# Autodesk Inventor assembly: planetaryGearBox
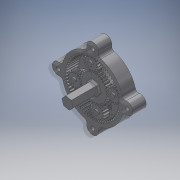
[picture p0: Inventor's stored thumbnail of the model, 180x180]
Saved by Autodesk Inventor 2019 (Build 230136000, 136)
## iProperties
Created: 2019-10-26
Part Number: planetaryGearBox
Document SubType Name: Assembly
Designer: test
Author: test
## Documents named in this file (6)
- C:\Users\test\Downloads\planetaryGearBox.iam
- C:\Users\test\Downloads\topPlateGB.ipt
- C:\Users\test\Downloads\planetaryGearMt2.ipt
- C:\Users\test\Downloads\RushGears_AP214_F3216.ipt
- C:\Users\test\Downloads\RushGears_AP214_F3232B.ipt
- C:\Users\test\Downloads\RushGears_AP214_F3264A.ipt
## Components (8 placed, 5 different names)
1. planetaryGearMt2:1 — Mate:1, Mate:2, Mate:3, Mate:4, Mate:5, Mate:6, Mate:7, Mate:8, Mate:10
2. RushGears_AP214_F3216:1 — Mate:3, Flush:1
3. RushGears_AP214_F3216:2 — Mate:5, Flush:4
4. RushGears_AP214_F3216:3 — Mate:6, Flush:2
5. RushGears_AP214_F3216:4 — Mate:4, Flush:3
6. RushGears_AP214_F3232B:1 — Mate:7, Flush:1, Flush:2, Flush:3, Flush:4, Mate:8
7. RushGears_AP214_F3264A:1 — Mate:1, Mate:2, Mate:9, Mate:11
8. topPlateGB:2 — Mate:9, Mate:10, Mate:11
## Relationships (15: Mate 11, Flush 4)
- Mate:1: planetaryGearMt2:1 ↔ RushGears_AP214_F3264A:1
- Mate:2: planetaryGearMt2:1 ↔ RushGears_AP214_F3264A:1
- Mate:3: planetaryGearMt2:1 ↔ RushGears_AP214_F3216:1
- Mate:4: planetaryGearMt2:1 ↔ RushGears_AP214_F3216:4
- Mate:5: planetaryGearMt2:1 ↔ RushGears_AP214_F3216:2
- Mate:6: planetaryGearMt2:1 ↔ RushGears_AP214_F3216:3
- Mate:7: planetaryGearMt2:1 ↔ RushGears_AP214_F3232B:1
- Flush:1: RushGears_AP214_F3216:1 ↔ RushGears_AP214_F3232B:1
- Flush:2: RushGears_AP214_F3216:3 ↔ RushGears_AP214_F3232B:1
- Flush:3: RushGears_AP214_F3216:4 ↔ RushGears_AP214_F3232B:1
- Flush:4: RushGears_AP214_F3216:2 ↔ RushGears_AP214_F3232B:1
- Mate:8: planetaryGearMt2:1 ↔ RushGears_AP214_F3232B:1
- Mate:9: RushGears_AP214_F3264A:1 ↔ topPlateGB:2
- Mate:10: planetaryGearMt2:1 ↔ topPlateGB:2
- Mate:11: RushGears_AP214_F3264A:1 ↔ topPlateGB:2
